# Autodesk Inventor assembly: Interior Elevator
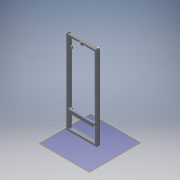
[picture p0: Inventor's stored thumbnail of the model, 180x180]
Saved by Autodesk Inventor 2018 (Build 220112000, 112)
## iProperties
Created: 2015-12-07
Part Number: Interior Elevator
Description: STEP AP214
Document SubType Name: Assembly
Designer: brooksprench
Sending System: SolidWorks 2014
Preprocessor: SwSTEP 2.0
Title: AM14U3 Square REV1-1.STEP
Revision Number: ANY
## Documents named in this file (8)
- C:\Users\uzair\Documents\School\Clubs\Robotics\CAD for Unity\Interior Elevator.iam
- C:\Users\uzair\Documents\School\Clubs\Robotics\2018Robot\4992 Robot v0.1\4992-2018-Elvator-Interior Bottom Rail.ipt
- C:\Users\uzair\Documents\School\Clubs\Robotics\2018Robot\4992 Robot v0.1\4992-2018-Elvator-Inner Side Rail.ipt
- C:\Users\uzair\Documents\School\Clubs\Robotics\2018Robot\4992 Robot v0.1\4992-2018-Elvator-Interior Top Rail.ipt
- C:\Users\uzair\Documents\School\Clubs\Robotics\2018Robot\4992 Robot v0.1\4992-2018-Elvator-Interior WS_16_Rail.ipt
- C:\Users\uzair\Documents\School\Clubs\Robotics\2018Robot\4992 Robot v0.1\4992-2018-Elvator-Interior WE7UM_Bearing_Block.ipt
- C:\Users\uzair\Documents\School\Clubs\Robotics\2018Robot\4992 Robot v0.1\4992-2018-Elvator-Interior Carriage Plate.ipt
- C:\Users\uzair\Documents\School\Clubs\Robotics\2018Robot\4992 Robot v0.1\3071T100_MOUNTED PULLEY FOR FIBROUS ROPE.ipt
## Components (11 placed, 7 different names)
1. 4992-2018-Elvator-Interior Bottom Rail:1 — Mate:15, Mate:17, Flush:10, Mate:18, Flush:11
2. 4992-2018-Elvator-Inner Side Rail:1 — Mate:17, Mate:18, Flush:11, Mate:19, Mate:22, Flush:14
3. 4992-2018-Elvator-Inner Side Rail:2 — Mate:15, Flush:10, Mate:20, Flush:12, Flush:13, Mate:21, Flush:15, Flush:20
4. 4992-2018-Elvator-Interior Top Rail:1 — Mate:19, Mate:20, Flush:12, Flush:13, Mate:23, Mate:24, Mate:28
5. 4992-2018-Elvator-Interior WS_16_Rail:1 — Mate:21, Mate:23, Flush:15, Cylindrical:3
6. 4992-2018-Elvator-Interior WS_16_Rail:2 — Mate:22, Mate:24, Cylindrical:1, Flush:14, Cylindrical:2
7. 4992-2018-Elvator-Interior WE7UM_Bearing_Block:1 — Cylindrical:2, Mate:25, Flush:16, Flush:18
8. 4992-2018-Elvator-Interior WE7UM_Bearing_Block:2 — Cylindrical:3, Mate:26, Flush:17
9. 4992-2018-Elvator-Interior WE7UM_Bearing_Block:3 — Cylindrical:1
10. 4992-2018-Elvator-Interior Carriage Plate:1 — Mate:25, Mate:26, Flush:16, Flush:17, Flush:18
11. 3071T100_MOUNTED PULLEY FOR FIBROUS ROPE:1 — Flush:20, Mate:28
## Relationships (25: Mate 12, Flush 10, CylindricalJoint 3)
- Mate:15: 4992-2018-Elvator-Interior Bottom Rail:1 ↔ 4992-2018-Elvator-Inner Side Rail:2
- Mate:17: 4992-2018-Elvator-Interior Bottom Rail:1 ↔ 4992-2018-Elvator-Inner Side Rail:1
- Flush:10: 4992-2018-Elvator-Interior Bottom Rail:1 ↔ 4992-2018-Elvator-Inner Side Rail:2
- Mate:18: 4992-2018-Elvator-Interior Bottom Rail:1 ↔ 4992-2018-Elvator-Inner Side Rail:1
- Flush:11: 4992-2018-Elvator-Interior Bottom Rail:1 ↔ 4992-2018-Elvator-Inner Side Rail:1
- Mate:19: 4992-2018-Elvator-Inner Side Rail:1 ↔ 4992-2018-Elvator-Interior Top Rail:1
- Mate:20: 4992-2018-Elvator-Inner Side Rail:2 ↔ 4992-2018-Elvator-Interior Top Rail:1
- Flush:12: 4992-2018-Elvator-Inner Side Rail:2 ↔ 4992-2018-Elvator-Interior Top Rail:1
- Flush:13: 4992-2018-Elvator-Inner Side Rail:2 ↔ 4992-2018-Elvator-Interior Top Rail:1
- Mate:21: 4992-2018-Elvator-Inner Side Rail:2 ↔ 4992-2018-Elvator-Interior WS_16_Rail:1
- Mate:22: 4992-2018-Elvator-Inner Side Rail:1 ↔ 4992-2018-Elvator-Interior WS_16_Rail:2
- Mate:23: 4992-2018-Elvator-Interior Top Rail:1 ↔ 4992-2018-Elvator-Interior WS_16_Rail:1
- Mate:24: 4992-2018-Elvator-Interior Top Rail:1 ↔ 4992-2018-Elvator-Interior WS_16_Rail:2
- Cylindrical:1: 4992-2018-Elvator-Interior WS_16_Rail:2 ↔ 4992-2018-Elvator-Interior WE7UM_Bearing_Block:3
- Flush:14: 4992-2018-Elvator-Inner Side Rail:1 ↔ 4992-2018-Elvator-Interior WS_16_Rail:2
- Flush:15: 4992-2018-Elvator-Inner Side Rail:2 ↔ 4992-2018-Elvator-Interior WS_16_Rail:1
- Cylindrical:2: 4992-2018-Elvator-Interior WS_16_Rail:2 ↔ 4992-2018-Elvator-Interior WE7UM_Bearing_Block:1
- Cylindrical:3: 4992-2018-Elvator-Interior WS_16_Rail:1 ↔ 4992-2018-Elvator-Interior WE7UM_Bearing_Block:2
- Mate:25: 4992-2018-Elvator-Interior WE7UM_Bearing_Block:1 ↔ 4992-2018-Elvator-Interior Carriage Plate:1
- Mate:26: 4992-2018-Elvator-Interior WE7UM_Bearing_Block:2 ↔ 4992-2018-Elvator-Interior Carriage Plate:1
- Flush:16: 4992-2018-Elvator-Interior WE7UM_Bearing_Block:1 ↔ 4992-2018-Elvator-Interior Carriage Plate:1
- Flush:17: 4992-2018-Elvator-Interior WE7UM_Bearing_Block:2 ↔ 4992-2018-Elvator-Interior Carriage Plate:1
- Flush:18: 4992-2018-Elvator-Interior WE7UM_Bearing_Block:1 ↔ 4992-2018-Elvator-Interior Carriage Plate:1
- Flush:20 (215.9 mm): 4992-2018-Elvator-Inner Side Rail:2 ↔ 3071T100_MOUNTED PULLEY FOR FIBROUS ROPE:1
- Mate:28: 4992-2018-Elvator-Interior Top Rail:1 ↔ 3071T100_MOUNTED PULLEY FOR FIBROUS ROPE:1
